# Autodesk Inventor assembly: ASY MSC 800 gills
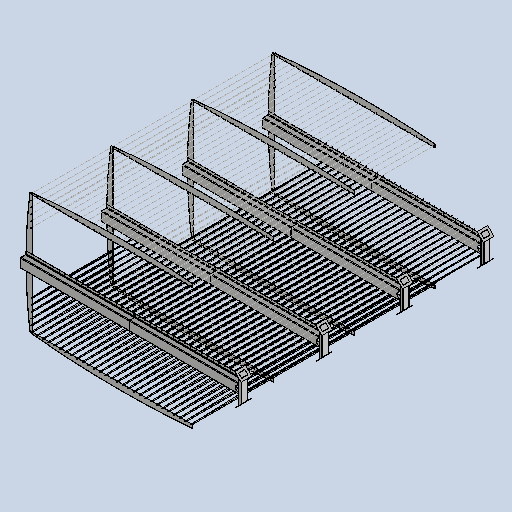
[picture p0: Inventor's stored thumbnail of the model, 512x512]
Saved by Autodesk Inventor 2025 (Build 290162010, 162A)
## iProperties
Created: 2024-08-31
Part Number: ASY MSC 800 gills
Document SubType Name: Assembly
Designer: pokla
Stock Number: ASY МОО 800 Жабры
Mass: 57918.9 g
Surface Area: 154099 cm^2
Volume: 7985.94 cm^3
Density: 7.25262 g/cm^3
Author: pokla
## Documents named in this file (14)
- C:\Users\admin\YandexDisk-badmisterfox\домашниий пк\Inventor\Manturovo\Manturovo_Se-clar\ASY MSC 800 gills.iam
- C:\Users\admin\YandexDisk-badmisterfox\домашниий пк\Inventor\Manturovo\Manturovo_Se-clar\MSC 804 sheet gills.ipt
- C:\Users\admin\YandexDisk-badmisterfox\домашниий пк\Inventor\Manturovo\Manturovo_Se-clar\MSC 810 pillar gills.ipt
- C:\Users\admin\YandexDisk-badmisterfox\домашниий пк\Inventor\Manturovo\Manturovo_Se-clar\MSC 805 sheet gills.ipt
- C:\Users\admin\YandexDisk-badmisterfox\домашниий пк\Inventor\Manturovo\Manturovo_Se-clar\MSC 806 sheet gills.ipt
- C:\Users\admin\YandexDisk-badmisterfox\домашниий пк\Inventor\Manturovo\Manturovo_Se-clar\MSC 807 sheet gills.ipt
- C:\Users\admin\YandexDisk-badmisterfox\домашниий пк\Inventor\Manturovo\Manturovo_Se-clar\MSC 808 sheet gills.ipt
- C:\Users\admin\YandexDisk-badmisterfox\домашниий пк\Inventor\Manturovo\Manturovo_Se-clar\MSC 809 sheet gills.ipt
- C:\Users\admin\YandexDisk-badmisterfox\домашниий пк\Inventor\Manturovo\Manturovo_Se-clar\MSC 813 wall support gills.ipt
- C:\Users\admin\YandexDisk-badmisterfox\домашниий пк\Inventor\Manturovo\Manturovo_Se-clar\MSC 811 pillar gills.ipt
- C:\Users\admin\YandexDisk-badmisterfox\домашниий пк\Inventor\Manturovo\Manturovo_Se-clar\MSC 814 string for sheets gills.ipt
- C:\Users\admin\YandexDisk-badmisterfox\домашниий пк\Inventor\Manturovo\Manturovo_Se-clar\MSC 812 top support gills.ipt
- C:\Users\admin\YandexDisk-badmisterfox\домашниий пк\Inventor\Manturovo\Manturovo_Se-clar\MSC 803 sheet gills.ipt
- C:\Users\admin\YandexDisk-badmisterfox\домашниий пк\Inventor\Manturovo\Manturovo_Se-clar\ASY MSC 800.1 gills base.iam
## Components (214 placed, 13 different names)
1. MSC 805 sheet gills.ipt:1 — Angle:2, Tangent:8, Tangent:9, Flush:15, Flush:19
2. MSC 806 sheet gills.ipt:1 — Angle:3, Tangent:10, Tangent:11, Flush:15, Flush:16
3. MSC 807 sheet gills.ipt:1 — Angle:4, Tangent:12, Tangent:13, Flush:16, Flush:17
4. MSC 808 sheet gills.ipt:1 — Angle:5, Tangent:17, Tangent:18, Flush:17, Flush:18
5. MSC 809 sheet gills.ipt:1 — Angle:6, Tangent:19, Tangent:20, Flush:18
6. MSC 814 string for sheets gills.ipt:1 — Rigid:40
7. MSC 814 string for sheets gills.ipt:2 — Rigid:24
8. MSC 814 string for sheets gills.ipt:3
9. MSC 814 string for sheets gills.ipt:4
10. MSC 814 string for sheets gills.ipt:5
11. MSC 814 string for sheets gills.ipt:6
12. MSC 814 string for sheets gills.ipt:7
13. MSC 814 string for sheets gills.ipt:8 — Rigid:12
14. MSC 803 sheet gills.ipt:1 — Rigid:33, Angle:2, Angle:3, Angle:4, Angle:5, Angle:6, Tangent:14, Tangent:15, Tangent:16, Flush:19
15. MSC 804 sheet gills.ipt:1 — Rigid:33
16. MSC 814 string for sheets gills.ipt:9 — Rotational:1
17. MSC 814 string for sheets gills.ipt:10 — Rotational:2
18. MSC 814 string for sheets gills.ipt:11 — Rotational:3
19. MSC 814 string for sheets gills.ipt:12
20. MSC 803 sheet gills.ipt:2
21. MSC 804 sheet gills.ipt:2
22. MSC 814 string for sheets gills.ipt:13
23. MSC 814 string for sheets gills.ipt:14
24. MSC 814 string for sheets gills.ipt:15
25. MSC 814 string for sheets gills.ipt:16
26. MSC 803 sheet gills.ipt:3
27. MSC 804 sheet gills.ipt:3
28. MSC 814 string for sheets gills.ipt:17
29. MSC 814 string for sheets gills.ipt:18
30. MSC 814 string for sheets gills.ipt:19
31. MSC 814 string for sheets gills.ipt:20
32. MSC 803 sheet gills.ipt:4
33. MSC 804 sheet gills.ipt:4
34. MSC 814 string for sheets gills.ipt:21
35. MSC 814 string for sheets gills.ipt:22
36. MSC 814 string for sheets gills.ipt:23
37. MSC 814 string for sheets gills.ipt:24
38. MSC 803 sheet gills.ipt:5
39. MSC 804 sheet gills.ipt:5
40. MSC 814 string for sheets gills.ipt:25
41. MSC 814 string for sheets gills.ipt:26
42. MSC 814 string for sheets gills.ipt:27
43. MSC 814 string for sheets gills.ipt:28
44. MSC 803 sheet gills.ipt:6
45. MSC 804 sheet gills.ipt:6
46. MSC 814 string for sheets gills.ipt:29
47. MSC 814 string for sheets gills.ipt:30
48. MSC 814 string for sheets gills.ipt:31
49. MSC 814 string for sheets gills.ipt:32
50. MSC 803 sheet gills.ipt:7
51. MSC 804 sheet gills.ipt:7
52. MSC 814 string for sheets gills.ipt:33
53. MSC 814 string for sheets gills.ipt:34
54. MSC 814 string for sheets gills.ipt:35
55. MSC 814 string for sheets gills.ipt:36
56. MSC 803 sheet gills.ipt:8
57. MSC 804 sheet gills.ipt:8
58. MSC 814 string for sheets gills.ipt:37
59. MSC 814 string for sheets gills.ipt:38
60. MSC 814 string for sheets gills.ipt:39
61. MSC 814 string for sheets gills.ipt:40
62. MSC 803 sheet gills.ipt:9
63. MSC 804 sheet gills.ipt:9
64. MSC 814 string for sheets gills.ipt:41
65. MSC 814 string for sheets gills.ipt:42
66. MSC 814 string for sheets gills.ipt:43
67. MSC 814 string for sheets gills.ipt:44
68. MSC 803 sheet gills.ipt:10
69. MSC 804 sheet gills.ipt:10
70. MSC 814 string for sheets gills.ipt:45
71. MSC 814 string for sheets gills.ipt:46
72. MSC 814 string for sheets gills.ipt:47
73. MSC 814 string for sheets gills.ipt:48
74. MSC 803 sheet gills.ipt:11
75. MSC 804 sheet gills.ipt:11
76. MSC 814 string for sheets gills.ipt:49
77. MSC 814 string for sheets gills.ipt:50
78. MSC 814 string for sheets gills.ipt:51
79. MSC 814 string for sheets gills.ipt:52
80. MSC 803 sheet gills.ipt:12
81. MSC 804 sheet gills.ipt:12
82. MSC 814 string for sheets gills.ipt:53
83. MSC 814 string for sheets gills.ipt:54
84. MSC 814 string for sheets gills.ipt:55
85. MSC 814 string for sheets gills.ipt:56
86. MSC 803 sheet gills.ipt:13
87. MSC 804 sheet gills.ipt:13
88. MSC 814 string for sheets gills.ipt:57
89. MSC 814 string for sheets gills.ipt:58
90. MSC 814 string for sheets gills.ipt:59
91. MSC 814 string for sheets gills.ipt:60
92. MSC 803 sheet gills.ipt:14
93. MSC 804 sheet gills.ipt:14
94. MSC 814 string for sheets gills.ipt:61
95. MSC 814 string for sheets gills.ipt:62
96. MSC 814 string for sheets gills.ipt:63
97. MSC 814 string for sheets gills.ipt:64
98. MSC 803 sheet gills.ipt:15
99. MSC 804 sheet gills.ipt:15
100. MSC 814 string for sheets gills.ipt:65
101. MSC 814 string for sheets gills.ipt:66
102. MSC 814 string for sheets gills.ipt:67
103. MSC 814 string for sheets gills.ipt:68
104. MSC 803 sheet gills.ipt:16
105. MSC 804 sheet gills.ipt:16
106. MSC 814 string for sheets gills.ipt:69
107. MSC 814 string for sheets gills.ipt:70
108. MSC 814 string for sheets gills.ipt:71
109. MSC 814 string for sheets gills.ipt:72
110. MSC 803 sheet gills.ipt:17
111. MSC 804 sheet gills.ipt:17
112. MSC 814 string for sheets gills.ipt:73
113. MSC 814 string for sheets gills.ipt:74
114. MSC 814 string for sheets gills.ipt:75
115. MSC 814 string for sheets gills.ipt:76
116. MSC 803 sheet gills.ipt:18
117. MSC 804 sheet gills.ipt:18
118. MSC 814 string for sheets gills.ipt:77
119. MSC 814 string for sheets gills.ipt:78
120. MSC 814 string for sheets gills.ipt:79
121. MSC 814 string for sheets gills.ipt:80
122. MSC 803 sheet gills.ipt:19
123. MSC 804 sheet gills.ipt:19
124. MSC 814 string for sheets gills.ipt:81
125. MSC 814 string for sheets gills.ipt:82
126. MSC 814 string for sheets gills.ipt:83
127. MSC 814 string for sheets gills.ipt:84
128. MSC 803 sheet gills.ipt:20
129. MSC 804 sheet gills.ipt:20
130. MSC 814 string for sheets gills.ipt:85
131. MSC 814 string for sheets gills.ipt:86
132. MSC 814 string for sheets gills.ipt:87
133. MSC 814 string for sheets gills.ipt:88
134. MSC 803 sheet gills.ipt:21
135. MSC 804 sheet gills.ipt:21
136. MSC 814 string for sheets gills.ipt:89
137. MSC 814 string for sheets gills.ipt:90
138. MSC 814 string for sheets gills.ipt:91
139. MSC 814 string for sheets gills.ipt:92
140. MSC 803 sheet gills.ipt:22
141. MSC 804 sheet gills.ipt:22
142. MSC 814 string for sheets gills.ipt:93
143. MSC 814 string for sheets gills.ipt:94
144. MSC 814 string for sheets gills.ipt:95
145. MSC 814 string for sheets gills.ipt:96
146. MSC 803 sheet gills.ipt:23
147. MSC 804 sheet gills.ipt:23
148. MSC 814 string for sheets gills.ipt:97
149. MSC 814 string for sheets gills.ipt:98
150. MSC 814 string for sheets gills.ipt:99
151. MSC 814 string for sheets gills.ipt:100
152. MSC 803 sheet gills.ipt:24
153. MSC 804 sheet gills.ipt:24
154. MSC 814 string for sheets gills.ipt:101
155. MSC 814 string for sheets gills.ipt:102
156. MSC 814 string for sheets gills.ipt:103
157. MSC 814 string for sheets gills.ipt:104
158. MSC 803 sheet gills.ipt:25
159. MSC 804 sheet gills.ipt:25
160. MSC 814 string for sheets gills.ipt:105
161. MSC 814 string for sheets gills.ipt:106
162. MSC 814 string for sheets gills.ipt:107
163. MSC 814 string for sheets gills.ipt:108
164. MSC 803 sheet gills.ipt:26
165. MSC 804 sheet gills.ipt:26
166. MSC 814 string for sheets gills.ipt:109
167. MSC 814 string for sheets gills.ipt:110
168. MSC 814 string for sheets gills.ipt:111
169. MSC 814 string for sheets gills.ipt:112
170. MSC 803 sheet gills.ipt:27
171. MSC 804 sheet gills.ipt:27
172. MSC 814 string for sheets gills.ipt:113
173. MSC 814 string for sheets gills.ipt:114
174. MSC 814 string for sheets gills.ipt:115
175. MSC 814 string for sheets gills.ipt:116
176. MSC 803 sheet gills.ipt:28
177. MSC 804 sheet gills.ipt:28
178. MSC 814 string for sheets gills.ipt:117
179. MSC 814 string for sheets gills.ipt:118
180. MSC 814 string for sheets gills.ipt:119
181. MSC 814 string for sheets gills.ipt:120
182. MSC 803 sheet gills.ipt:29
183. MSC 804 sheet gills.ipt:29
184. MSC 814 string for sheets gills.ipt:121
185. MSC 814 string for sheets gills.ipt:122
186. MSC 814 string for sheets gills.ipt:123
187. MSC 813 wall support gills.ipt:1 — Rigid:12, Rigid:30, Tangent:14, Tangent:15
188. MSC 812 top support gills.ipt:1 — Rigid:28, Rigid:30, Tangent:8, Tangent:9, Tangent:10, Tangent:11, Tangent:12, Tangent:13, Tangent:17, Tangent:18, Tangent:19, Tangent:20, Rigid:40
189. MSC 811 pillar gills.ipt:1 — Rigid:28, Rigid:29
190. MSC 812 top support gills.ipt:2 — Rigid:24, Rigid:29, Rigid:31
191. MSC 813 wall support gills.ipt:2 — Rigid:31, Rotational:3
192. MSC 810 pillar gills.ipt:1 — Rotational:1, Rotational:2, Tangent:16
193. ASY MSC 800.1 gills base.iam:1 [sub-assembly]
194. MSC 813 wall support gills.ipt:3
195. MSC 812 top support gills.ipt:3
196. MSC 811 pillar gills.ipt:2
197. MSC 812 top support gills.ipt:4
198. MSC 813 wall support gills.ipt:4
199. MSC 810 pillar gills.ipt:2
200. ASY MSC 800.1 gills base.iam:2 [sub-assembly]
201. MSC 813 wall support gills.ipt:5
202. MSC 812 top support gills.ipt:5
203. MSC 811 pillar gills.ipt:3
204. MSC 812 top support gills.ipt:6
205. MSC 813 wall support gills.ipt:6
206. MSC 810 pillar gills.ipt:3
207. ASY MSC 800.1 gills base.iam:3 [sub-assembly]
208. MSC 813 wall support gills.ipt:7
209. MSC 812 top support gills.ipt:7
210. MSC 811 pillar gills.ipt:4
211. MSC 812 top support gills.ipt:8
212. MSC 813 wall support gills.ipt:8
213. MSC 810 pillar gills.ipt:4
214. ASY MSC 800.1 gills base.iam:4 [sub-assembly]
## Component patterns: (6 elements, first: MSC 814 string for sheets gills.ipt:2), (29 elements, first: MSC 814 string for sheets gills.ipt:8 + MSC 803 sheet gills.ipt:1 + MSC 804 sheet gills.ipt:1 + MSC 814 string for sheets gills.ipt:9 + MSC 814 string for sheets gills.ipt:10 + MSC 814 string for sheets gills.ipt:11), (4 elements, first: MSC 813 wall support gills.ipt:1 + MSC 812 top support gills.ipt:1 + MSC 811 pillar gills.ipt:1 + MSC 812 top support gills.ipt:2 + MSC 813 wall support gills.ipt:2 + MSC 810 pillar gills.ipt:1 + ASY MSC 800.1 gills base.iam:1)
## Relationships (41: Tangent 13, WeldJoint 9, Flush 8, Angle 5, Mate 3, RevoluteJoint 3)
- [WeldJoint]: MSC 811 pillar gills.ipt:1 ↔ MSC 810 pillar gills.ipt:1
- [Flush]: MSC 810 pillar gills.ipt:1 ↔ ASY MSC 800.1 gills base.iam:1
- [Mate]: MSC 810 pillar gills.ipt:1 ↔ ASY MSC 800.1 gills base.iam:1
- [Flush] (5 mm): MSC 810 pillar gills.ipt:1 ↔ ASY MSC 800.1 gills base.iam:1
- Rigid:12 [WeldJoint] (-5 mm): MSC 814 string for sheets gills.ipt:8 ↔ MSC 813 wall support gills.ipt:1
- [Mate]: ASY MSC 800.1 gills base.iam:1
- [Mate]: ASY MSC 800.1 gills base.iam:1
- [Flush]: ASY MSC 800.1 gills base.iam:1
- Rigid:24 [WeldJoint] (-5 mm): MSC 814 string for sheets gills.ipt:2 ↔ MSC 812 top support gills.ipt:2
- Rigid:28 [WeldJoint]: MSC 812 top support gills.ipt:1 ↔ MSC 811 pillar gills.ipt:1
- Rigid:29 [WeldJoint]: MSC 811 pillar gills.ipt:1 ↔ MSC 812 top support gills.ipt:2
- Rigid:30 [WeldJoint]: MSC 813 wall support gills.ipt:1 ↔ MSC 812 top support gills.ipt:1
- Rigid:31 [WeldJoint]: MSC 812 top support gills.ipt:2 ↔ MSC 813 wall support gills.ipt:2
- Rotational:1 [RevoluteJoint] (5 mm): MSC 814 string for sheets gills.ipt:9 ↔ MSC 810 pillar gills.ipt:1
- Rotational:2 [RevoluteJoint] (-5 mm): MSC 814 string for sheets gills.ipt:10 ↔ MSC 810 pillar gills.ipt:1
- Rigid:33 [WeldJoint] (-10 mm): MSC 803 sheet gills.ipt:1 ↔ MSC 804 sheet gills.ipt:1
- Angle:2 (0 deg): MSC 805 sheet gills.ipt:1 ↔ MSC 803 sheet gills.ipt:1
- Angle:3 (0 deg): MSC 806 sheet gills.ipt:1 ↔ MSC 803 sheet gills.ipt:1
- Angle:4 (0 deg): MSC 807 sheet gills.ipt:1 ↔ MSC 803 sheet gills.ipt:1
- Angle:5 (0 deg): MSC 808 sheet gills.ipt:1 ↔ MSC 803 sheet gills.ipt:1
- Angle:6 (0 deg): MSC 809 sheet gills.ipt:1 ↔ MSC 803 sheet gills.ipt:1
- Tangent:8: MSC 805 sheet gills.ipt:1 ↔ MSC 812 top support gills.ipt:1
- Tangent:9: MSC 805 sheet gills.ipt:1 ↔ MSC 812 top support gills.ipt:1
- Tangent:10: MSC 806 sheet gills.ipt:1 ↔ MSC 812 top support gills.ipt:1
- Tangent:11: MSC 806 sheet gills.ipt:1 ↔ MSC 812 top support gills.ipt:1
- Tangent:12: MSC 807 sheet gills.ipt:1 ↔ MSC 812 top support gills.ipt:1
- Tangent:13: MSC 807 sheet gills.ipt:1 ↔ MSC 812 top support gills.ipt:1
- Tangent:14: MSC 803 sheet gills.ipt:1 ↔ MSC 813 wall support gills.ipt:1
- Tangent:15: MSC 803 sheet gills.ipt:1 ↔ MSC 813 wall support gills.ipt:1
- Tangent:16: MSC 803 sheet gills.ipt:1 ↔ MSC 810 pillar gills.ipt:1
- Tangent:17: MSC 808 sheet gills.ipt:1 ↔ MSC 812 top support gills.ipt:1
- Tangent:18: MSC 808 sheet gills.ipt:1 ↔ MSC 812 top support gills.ipt:1
- Tangent:19: MSC 809 sheet gills.ipt:1 ↔ MSC 812 top support gills.ipt:1
- Tangent:20: MSC 809 sheet gills.ipt:1 ↔ MSC 812 top support gills.ipt:1
- Flush:15: MSC 805 sheet gills.ipt:1 ↔ MSC 806 sheet gills.ipt:1
- Flush:16: MSC 806 sheet gills.ipt:1 ↔ MSC 807 sheet gills.ipt:1
- Flush:17: MSC 807 sheet gills.ipt:1 ↔ MSC 808 sheet gills.ipt:1
- Flush:18: MSC 808 sheet gills.ipt:1 ↔ MSC 809 sheet gills.ipt:1
- Flush:19: MSC 805 sheet gills.ipt:1 ↔ MSC 803 sheet gills.ipt:1
- Rigid:40 [WeldJoint] (5 mm): MSC 814 string for sheets gills.ipt:1 ↔ MSC 812 top support gills.ipt:1
- Rotational:3 [RevoluteJoint] (-5 mm): MSC 814 string for sheets gills.ipt:11 ↔ MSC 813 wall support gills.ipt:2
